# Autodesk Inventor assembly: layers3-6
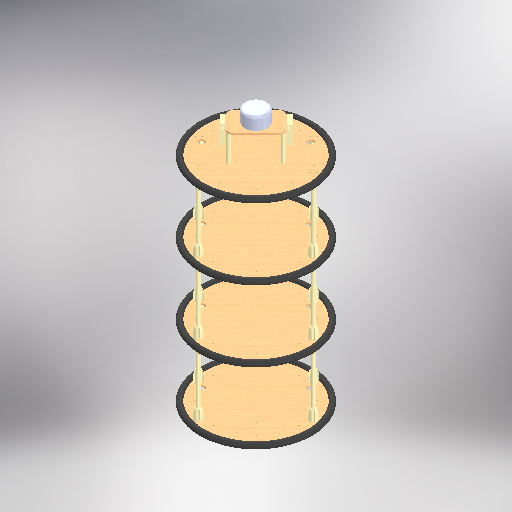
[picture p0: Inventor's stored thumbnail of the model, 512x512]
Saved by Autodesk Inventor 2026 (Build 300175050, 175E)
## iProperties
Created: 2025-08-11
Part Number: layers3-6
Document SubType Name: Assembly
Designer: satom
Author: satom
## Documents named in this file (20)
- C:\Users\satom\Desktop\Robot\CAD\Inventor\layers3-6.iam
- C:\Users\satom\Desktop\Robot\CAD\Inventor\C - Chassis\layer3_new.ipt
- C:\Users\satom\Desktop\Robot\CAD\Inventor\C - Chassis\9inch_spacer.ipt
- C:\Users\satom\Desktop\Robot\CAD\Inventor\C - Chassis\layer4_new.ipt
- C:\Users\satom\Desktop\Robot\CAD\Inventor\C - Chassis\layer5_new.ipt
- C:\Users\satom\Desktop\Robot\CAD\Inventor\C - Chassis\layer6_new.ipt
- C:\Users\satom\Desktop\Robot\CAD\Inventor\C - Chassis\3.5inch_standoff.ipt
- C:\Users\satom\Desktop\Robot\CAD\Inventor\solidworks\Display\Arducam_assembly\Arducam_assembly\Arducam_assembly.ipt
- C:\Users\satom\Desktop\Robot\CAD\Inventor\C - Chassis\LiDAR_plate.ipt
- C:\Users\satom\Desktop\Robot\CAD\Inventor\solidworks\E - Electronics\A2_LIDAR\A2_LIDAR\A2_LIDAR.ipt
- C:\Users\satom\Desktop\Robot\CAD\Inventor\E - Electronics\microphone_casing.ipt
- C:\Users\satom\Desktop\Robot\CAD\Inventor\E - Electronics\microphone_casing_back.ipt
- C:\Users\satom\Desktop\Robot\CAD\Inventor\C - Chassis\display_top_support_left.ipt
- C:\Users\satom\Desktop\Robot\CAD\Inventor\C - Chassis\display_top_support_right.ipt
- C:\Users\satom\Desktop\Robot\CAD\Inventor\solidworks\Display\monitor\monitor\monitor.ipt
- C:\Users\satom\Desktop\Robot\CAD\Inventor\C - Chassis\display_bottom_support_left.ipt
- C:\Users\satom\Desktop\Robot\CAD\Inventor\C - Chassis\display_bottom_support_right.ipt
- C:\Users\satom\Desktop\Robot\CAD\Inventor\E - Electronics\astra_holder.ipt
- C:\Users\satom\Desktop\Robot\CAD\Inventor\C - Chassis\foam_bumper_circular.ipt
- C:\Users\satom\Desktop\Robot\CAD\Inventor\E - Electronics\astra_camera.ipt
## Components (38 placed, 19 different names)
1. layer3_new:1
2. 9inch_spacer:1
3. 9inch_spacer:2
4. 9inch_spacer:3
5. 9inch_spacer:4
6. layer4_new:1
7. 9inch_spacer:5
8. 9inch_spacer:6
9. 9inch_spacer:7
10. 9inch_spacer:8
11. layer5_new:1
12. 9inch_spacer:9
13. 9inch_spacer:10
14. 9inch_spacer:11
15. 9inch_spacer:12
16. layer6_new:1 — Mate:136, Mate:137
17. 3.5inch_standoff:1
18. 3.5inch_standoff:2
19. 3.5inch_standoff:3
20. 3.5inch_standoff:4
21. Arducam_assembly:1
22. LiDAR_plate:1
23. A2_LIDAR:1
24. microphone_casing:1 — Mate:136
25. microphone_casing_back:1
26. microphone_casing:2 — Mate:137
27. microphone_casing_back:2
28. display_top_support_left:1
29. display_top_support_right:1
30. monitor:1
31. display_bottom_support_left:1
32. display_bottom_support_right:1
33. astra_holder:1 — Mate:138
34. foam_bumper_circular:1
35. foam_bumper_circular:2
36. foam_bumper_circular:3
37. foam_bumper_circular:4
38. astra_camera:1 — Mate:138
## Relationships (139: Mate 138, Flush 1)
- [Mate]: layer3_new:1 ↔ 9inch_spacer:1
- [Mate]: layer3_new:1 ↔ 9inch_spacer:2
- [Mate]: layer3_new:1 ↔ 9inch_spacer:3
- [Mate]: layer3_new:1 ↔ 9inch_spacer:4
- [Mate]: layer3_new:1 ↔ 9inch_spacer:3
- [Mate]: layer3_new:1 ↔ 9inch_spacer:3
- [Mate]: layer3_new:1 ↔ 9inch_spacer:3
- [Mate]: layer3_new:1 ↔ 9inch_spacer:4
- [Mate]: layer3_new:1 ↔ 9inch_spacer:4
- [Mate]: layer3_new:1 ↔ 9inch_spacer:4
- [Mate]: layer3_new:1 ↔ 9inch_spacer:1
- [Mate]: layer3_new:1 ↔ 9inch_spacer:1
- [Mate]: layer3_new:1 ↔ 9inch_spacer:1
- [Mate]: layer3_new:1 ↔ 9inch_spacer:2
- [Mate]: layer3_new:1 ↔ 9inch_spacer:2
- [Mate]: layer3_new:1 ↔ 9inch_spacer:2
- [Mate]: 9inch_spacer:2 ↔ layer4_new:1
- [Mate]: 9inch_spacer:2 ↔ layer4_new:1
- [Mate]: 9inch_spacer:2 ↔ layer4_new:1
- [Mate]: 9inch_spacer:2 ↔ layer4_new:1
- [Mate]: 9inch_spacer:1 ↔ layer4_new:1
- [Mate]: 9inch_spacer:1 ↔ layer4_new:1
- [Mate]: 9inch_spacer:4 ↔ layer4_new:1
- [Mate]: 9inch_spacer:4 ↔ layer4_new:1
- [Mate]: 9inch_spacer:3 ↔ layer4_new:1
- [Mate]: 9inch_spacer:3 ↔ layer4_new:1
- [Mate]: layer4_new:1 ↔ 9inch_spacer:8
- [Mate]: layer4_new:1 ↔ 9inch_spacer:7
- [Mate]: layer4_new:1 ↔ 9inch_spacer:6
- [Mate]: layer4_new:1 ↔ 9inch_spacer:5
- [Mate]: layer4_new:1 ↔ 9inch_spacer:7
- [Mate]: layer4_new:1 ↔ 9inch_spacer:7
- [Mate]: layer4_new:1 ↔ 9inch_spacer:7
- [Mate]: layer4_new:1 ↔ 9inch_spacer:8
- [Mate]: layer4_new:1 ↔ 9inch_spacer:8
- [Mate]: layer4_new:1 ↔ 9inch_spacer:8
- [Mate]: layer4_new:1 ↔ 9inch_spacer:6
- [Mate]: layer4_new:1 ↔ 9inch_spacer:6
- [Mate]: layer4_new:1 ↔ 9inch_spacer:6
- [Mate]: layer4_new:1 ↔ 9inch_spacer:5
- [Mate]: layer4_new:1 ↔ 9inch_spacer:5
- [Mate]: layer4_new:1 ↔ 9inch_spacer:5
- [Mate]: 9inch_spacer:5 ↔ layer5_new:1
- [Mate]: 9inch_spacer:8 ↔ layer5_new:1
- [Mate]: 9inch_spacer:8 ↔ layer5_new:1
- [Mate]: 9inch_spacer:8 ↔ layer5_new:1
- [Mate]: 9inch_spacer:5 ↔ layer5_new:1
- [Mate]: 9inch_spacer:5 ↔ layer5_new:1
- [Mate]: 9inch_spacer:5 ↔ layer5_new:1
- [Mate]: 9inch_spacer:6 ↔ layer5_new:1
- [Mate]: 9inch_spacer:6 ↔ layer5_new:1
- [Mate]: 9inch_spacer:6 ↔ layer5_new:1
- [Mate]: 9inch_spacer:7 ↔ layer5_new:1
- [Mate]: 9inch_spacer:7 ↔ layer5_new:1
- [Mate]: 9inch_spacer:7 ↔ layer5_new:1
- [Mate]: layer5_new:1 ↔ 9inch_spacer:9
- [Mate]: layer5_new:1 ↔ 9inch_spacer:10
- [Mate]: layer5_new:1 ↔ 9inch_spacer:11
- [Mate]: layer5_new:1 ↔ 9inch_spacer:12
- [Mate]: layer5_new:1 ↔ 9inch_spacer:12
- [Mate]: layer5_new:1 ↔ 9inch_spacer:12
- [Mate]: layer5_new:1 ↔ 9inch_spacer:12
- [Mate]: layer5_new:1 ↔ 9inch_spacer:11
- [Mate]: layer5_new:1 ↔ 9inch_spacer:11
- [Mate]: layer5_new:1 ↔ 9inch_spacer:11
- [Mate]: layer5_new:1 ↔ 9inch_spacer:9
- [Mate]: layer5_new:1 ↔ 9inch_spacer:9
- [Mate]: layer5_new:1 ↔ 9inch_spacer:9
- [Mate]: layer5_new:1 ↔ 9inch_spacer:10
- [Mate]: layer5_new:1 ↔ 9inch_spacer:10
- [Mate]: layer5_new:1 ↔ 9inch_spacer:10
- [Mate]: 9inch_spacer:9 ↔ layer6_new:1
- [Mate]: 9inch_spacer:9 ↔ layer6_new:1
- [Mate]: 9inch_spacer:9 ↔ layer6_new:1
- [Mate]: 9inch_spacer:9 ↔ layer6_new:1
- [Mate]: 9inch_spacer:10 ↔ layer6_new:1
- [Mate]: 9inch_spacer:10 ↔ layer6_new:1
- [Mate]: 9inch_spacer:10 ↔ layer6_new:1
- [Mate]: 9inch_spacer:12 ↔ layer6_new:1
- [Mate]: 9inch_spacer:12 ↔ layer6_new:1
- [Mate]: 9inch_spacer:12 ↔ layer6_new:1
- [Mate]: 9inch_spacer:11 ↔ layer6_new:1
- [Mate]: 9inch_spacer:11 ↔ layer6_new:1
- [Mate]: 9inch_spacer:11 ↔ layer6_new:1
- [Mate]: layer6_new:1 ↔ 3.5inch_standoff:2
- [Mate]: layer6_new:1 ↔ 3.5inch_standoff:1
- [Mate]: layer6_new:1 ↔ 3.5inch_standoff:3
- [Mate]: layer6_new:1 ↔ 3.5inch_standoff:4
- [Mate]: layer6_new:1 ↔ 3.5inch_standoff:1
- [Mate]: layer6_new:1 ↔ 3.5inch_standoff:4
- [Mate]: layer6_new:1 ↔ 3.5inch_standoff:3
- [Mate]: layer6_new:1 ↔ 3.5inch_standoff:2
- [Mate]: layer6_new:1 ↔ Arducam_assembly:1
- [Mate]: layer6_new:1 ↔ Arducam_assembly:1
- [Mate]: 3.5inch_standoff:3 ↔ LiDAR_plate:1
- [Mate]: 3.5inch_standoff:1 ↔ LiDAR_plate:1
- [Mate]: 3.5inch_standoff:4 ↔ LiDAR_plate:1
- [Mate]: 3.5inch_standoff:2 ↔ LiDAR_plate:1
- [Mate]: 3.5inch_standoff:3 ↔ LiDAR_plate:1
- [Mate]: LiDAR_plate:1 ↔ A2_LIDAR:1
- [Mate]: LiDAR_plate:1 ↔ A2_LIDAR:1
- [Mate]: LiDAR_plate:1 ↔ A2_LIDAR:1
- [Mate]: LiDAR_plate:1 ↔ A2_LIDAR:1
- [Mate]: LiDAR_plate:1 ↔ A2_LIDAR:1
- [Mate]: microphone_casing:1 ↔ microphone_casing_back:1
- [Mate]: microphone_casing:1 ↔ microphone_casing_back:1
- [Mate]: microphone_casing:1 ↔ microphone_casing_back:1
- [Mate]: microphone_casing:2 ↔ microphone_casing_back:2
- [Mate]: microphone_casing:2 ↔ microphone_casing_back:2
- [Mate]: microphone_casing:2 ↔ microphone_casing_back:2
- [Mate]: 9inch_spacer:10 ↔ microphone_casing_back:1
- [Mate]: 9inch_spacer:9 ↔ microphone_casing_back:2
- [Mate]: layer6_new:1 ↔ display_top_support_left:1
- [Mate]: layer6_new:1 ↔ display_top_support_left:1
- [Mate]: layer6_new:1 ↔ display_top_support_right:1
- [Mate]: layer6_new:1 ↔ display_top_support_right:1
- [Mate]: display_top_support_right:1 ↔ monitor:1
- [Mate]: display_top_support_left:1 ↔ monitor:1
- [Mate]: layer6_new:1 ↔ display_bottom_support_left:1
- [Mate]: display_top_support_right:1 ↔ monitor:1
- [Mate]: monitor:1 ↔ display_bottom_support_left:1
- [Mate]: layer6_new:1 ↔ display_bottom_support_right:1
- [Mate]: monitor:1 ↔ display_bottom_support_right:1
- [Mate]: layer6_new:1 ↔ astra_holder:1
- [Mate]: layer6_new:1 ↔ astra_holder:1
- [Mate]: layer6_new:1 ↔ astra_holder:1
- [Mate]: layer3_new:1 ↔ foam_bumper_circular:1
- [Mate]: layer3_new:1 ↔ foam_bumper_circular:1
- [Mate]: layer4_new:1 ↔ foam_bumper_circular:2
- [Mate]: layer4_new:1 ↔ foam_bumper_circular:2
- [Mate]: layer5_new:1 ↔ foam_bumper_circular:3
- [Mate]: layer5_new:1 ↔ foam_bumper_circular:3
- [Mate]: layer6_new:1 ↔ foam_bumper_circular:4
- [Mate]: layer6_new:1 ↔ foam_bumper_circular:4
- [Mate]: astra_holder:1 ↔ astra_camera:1
- [Flush]: astra_holder:1 ↔ astra_camera:1
- Mate:136 (76.2 mm): layer6_new:1 ↔ microphone_casing:1
- Mate:137 (76.2 mm): layer6_new:1 ↔ microphone_casing:2
- Mate:138 (27.94 mm): astra_holder:1 ↔ astra_camera:1
## Named parameters: d81_d132 = 0 mm, d82_d133 = 0 mm, d83_d134 = 0 mm, d84_d135 = 0 mm
